# Autodesk Inventor assembly: capstone assembly
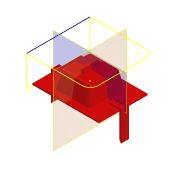
[picture p0: Inventor's stored thumbnail of the model, 180x180]
Saved by Autodesk Inventor 2020 (Build 240168000, 168)
## iProperties
Created: 2020-02-10
Part Number: capstone assembly
Document SubType Name: Assembly
Designer: ball
Author: ball
## Documents named in this file (3)
- C:\FTC\FTC8863CAD\2019 Robot\Delivery\Capstone\capstone assembly.iam
- C:\FTC\FTC8863CAD\2019 Robot\Delivery\Capstone\8863 capstone.3.ipt
- C:\FTC\FTC8863CAD\2019 Robot\Delivery\Capstone\capstone ear.ipt
## Components (3 placed, 2 different names)
1. 8863 capstone.3:1 — Mate:1, Mate:2, Mate:3, Mate:4, Mate:5, Mate:6
2. capstone ear:1 — Mate:4, Mate:5, Mate:6
3. capstone ear:2 — Mate:1, Mate:2, Mate:3
## Relationships (6: Mate 6)
- Mate:1: 8863 capstone.3:1 ↔ capstone ear:2
- Mate:2: 8863 capstone.3:1 ↔ capstone ear:2
- Mate:3: 8863 capstone.3:1 ↔ capstone ear:2
- Mate:4: 8863 capstone.3:1 ↔ capstone ear:1
- Mate:5: 8863 capstone.3:1 ↔ capstone ear:1
- Mate:6: 8863 capstone.3:1 ↔ capstone ear:1
